# Autodesk Inventor assembly: UBG-Dribbler v2
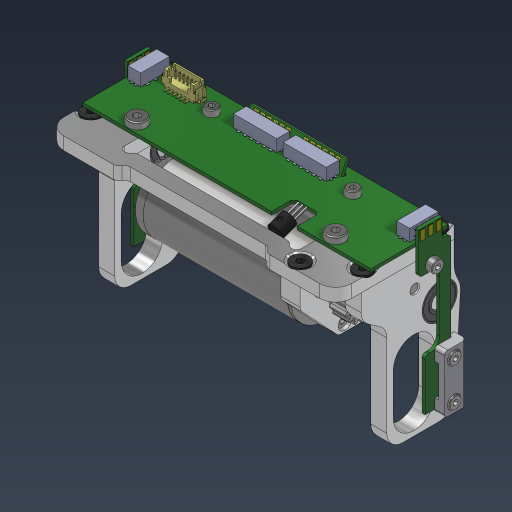
[picture p0: Inventor's stored thumbnail of the model, 512x512]
Saved by Autodesk Inventor 2023.1 (Build 271208000, 208)
## iProperties
RuleStatus: InUse
Part Number: UBG-Dribbler v2
Material: Generisch
Document SubType Name: Assembly
Designer: rYan
Mass: 217.02 g
Surface Area: 422.145 cm^2
Volume: 50.3668 cm^3
Author: rYan
## Documents named in this file (12)
- D:\TIGERsGIT\Hardware\mechanik\2024\Inventor\Robot\Dribbler\UBG-Dribbler v2.iam
- D:\TIGERsGIT\Hardware\mechanik\2024\Inventor\Robot\Dribbler\Dribbler Bruecke.ipt
- D:\TIGERsGIT\Hardware\mechanik\2024\Inventor\Robot\Electronics\MG-IR Empfänger.iam
- D:\TIGERsGIT\Hardware\mechanik\2024\Inventor\Robot\Electronics\MG-IR Sender.iam
- D:\TIGERsGIT\Hardware\mechanik\2024\Inventor\Robot\Electronics\MG-Ballsensor.iam
- D:\TIGERsGIT\Hardware\mechanik\2024\Inventor\Inhaltscenter\de-DE\ISO 4762(2)\ISO 4762 - M2 x 6ISO.ipt
- D:\TIGERsGIT\Hardware\mechanik\2024\Inventor\Inhaltscenter\de-DE\DIN 7984\DIN 7984 - M3 x 5.ipt
- D:\TIGERsGIT\Hardware\mechanik\2024\Inventor\Inhaltscenter\de-DE\ISO 10642(1)\ISO 10642 - M3 x  8.ipt
- D:\TIGERsGIT\Hardware\mechanik\2024\Inventor\Robot\Dribbler\MG-Dribbler Seite v2.iam
- D:\TIGERsGIT\Hardware\mechanik\2024\Inventor\Robot\Dribbler\MG-Dribblingwelle v2.iam
- D:\TIGERsGIT\Hardware\mechanik\2024\Inventor\Robot\Dribbler\MG-Dribblingmotor v2.iam
- D:\TIGERsGIT\Hardware\mechanik\2024\Inventor\Robot\Dribbler\MG-Dribbler Zwischenzahnrad v2.iam
## Components (23 placed, 11 different names)
1. Dribbler Bruecke:1 — Fluchtend:1, Passend:1, Fluchtend:2, Einfügen:1, Einfügen:2, Passend:2, Passend:3, Einfügen:8, Passend:21, Einfügen:10, Einfügen:11, Einfügen:12, Passend:24, Einfügen:13, Einfügen:14, Einfügen:15, Einfügen:16
2. MG-Dribbler Seite v2:3 [sub-assembly] — Einfügen:2, Passend:2, Einfügen:6, Passend:16
3. MG-Dribbler Seite v2:4 [sub-assembly] — Einfügen:1, Passend:3, Einfügen:7, Passend:17, Einfügen:25, Passend:25, Passend:28, Passend:29
4. MG-Dribblingwelle v2:1 [sub-assembly] — Passend:25, Passend:26
5. MG-Ballsensor:1 [sub-assembly] — Einfügen:8, Passend:21, Einfügen:23, Einfügen:24
6. MG-IR Empfänger:1 [sub-assembly] — Einfügen:7, Passend:17, Einfügen:18, Einfügen:21, Einfügen:22
7. MG-IR Sender:1 [sub-assembly] — Einfügen:6, Passend:16, Einfügen:17, Einfügen:19, Einfügen:20
8. ISO 10642 M3 x  8:1 — Einfügen:10
9. ISO 10642 M3 x  8:2 — Einfügen:11
10. MG-Dribblingmotor v2:1 [sub-assembly] — Einfügen:12, Passend:24
11. ISO 10642 M3 x  8:3 — Einfügen:13
12. ISO 10642 M3 x  8:4 — Einfügen:14
13. ISO 10642 M3 x  8:5 — Einfügen:15
14. ISO 10642 M3 x  8:6 — Einfügen:16
15. ISO 4762 M2 x 6:1 — Einfügen:17
16. ISO 4762 M2 x 6:2 — Einfügen:18
17. ISO 4762 M2 x 6:3 — Einfügen:19
18. ISO 4762 M2 x 6:4 — Einfügen:20
19. ISO 4762 M2 x 6:5 — Einfügen:22
20. ISO 4762 M2 x 6:6 — Einfügen:21
21. DIN 7984 M3 x 5:1 — Einfügen:23
22. DIN 7984 M3 x 5:2 — Einfügen:24
23. MG-Dribbler Zwischenzahnrad v2:1 [sub-assembly] — Einfügen:25
## Relationships (36: Insert 21, Mate 13, Flush 2)
- Fluchtend:1 [Flush]: Dribbler Bruecke:1
- Passend:1 [Mate]: Dribbler Bruecke:1
- Fluchtend:2 [Flush]: Dribbler Bruecke:1
- Einfügen:1 [Insert]: Dribbler Bruecke:1 ↔ MG-Dribbler Seite v2:4
- Einfügen:2 [Insert]: Dribbler Bruecke:1 ↔ MG-Dribbler Seite v2:3
- Passend:2 [Mate]: Dribbler Bruecke:1 ↔ MG-Dribbler Seite v2:3
- Passend:3 [Mate]: Dribbler Bruecke:1 ↔ MG-Dribbler Seite v2:4
- Einfügen:6 [Insert]: MG-Dribbler Seite v2:3 ↔ MG-IR Sender:1
- Passend:16 [Mate]: MG-Dribbler Seite v2:3 ↔ MG-IR Sender:1
- Einfügen:7 [Insert]: MG-Dribbler Seite v2:4 ↔ MG-IR Empfänger:1
- Passend:17 [Mate]: MG-Dribbler Seite v2:4 ↔ MG-IR Empfänger:1
- Einfügen:8 [Insert]: Dribbler Bruecke:1 ↔ MG-Ballsensor:1
- Passend:21 [Mate]: Dribbler Bruecke:1 ↔ MG-Ballsensor:1
- Einfügen:10 [Insert]: Dribbler Bruecke:1 ↔ ISO 10642 M3 x  8:1
- Einfügen:11 [Insert]: Dribbler Bruecke:1 ↔ ISO 10642 M3 x  8:2
- Einfügen:12 [Insert]: Dribbler Bruecke:1 ↔ MG-Dribblingmotor v2:1
- Passend:24 [Mate]: Dribbler Bruecke:1 ↔ MG-Dribblingmotor v2:1
- Einfügen:13 [Insert]: Dribbler Bruecke:1 ↔ ISO 10642 M3 x  8:3
- Einfügen:14 [Insert]: Dribbler Bruecke:1 ↔ ISO 10642 M3 x  8:4
- Einfügen:15 [Insert]: Dribbler Bruecke:1 ↔ ISO 10642 M3 x  8:5
- Einfügen:16 [Insert]: Dribbler Bruecke:1 ↔ ISO 10642 M3 x  8:6
- Einfügen:17 [Insert]: MG-IR Sender:1 ↔ ISO 4762 M2 x 6:1
- Einfügen:18 [Insert]: MG-IR Empfänger:1 ↔ ISO 4762 M2 x 6:2
- Einfügen:19 [Insert]: MG-IR Sender:1 ↔ ISO 4762 M2 x 6:3
- Einfügen:20 [Insert]: MG-IR Sender:1 ↔ ISO 4762 M2 x 6:4
- Einfügen:21 [Insert]: MG-IR Empfänger:1 ↔ ISO 4762 M2 x 6:6
- Einfügen:22 [Insert]: MG-IR Empfänger:1 ↔ ISO 4762 M2 x 6:5
- Einfügen:23 [Insert]: MG-Ballsensor:1 ↔ DIN 7984 M3 x 5:1
- Einfügen:24 [Insert]: MG-Ballsensor:1 ↔ DIN 7984 M3 x 5:2
- Einfügen:25 [Insert] (0.35 mm): MG-Dribbler Seite v2:4 ↔ MG-Dribbler Zwischenzahnrad v2:1
- Passend:25 [Mate]: MG-Dribbler Seite v2:4 ↔ MG-Dribblingwelle v2:1
- Passend:26 [Mate]: MG-Dribblingwelle v2:1
- Passend:28 [Mate]: MG-Dribbler Seite v2:4
- Passend:29 [Mate]: MG-Dribbler Seite v2:4
- Passend:30 [Mate]
- Passend:31 [Mate]
